# Autodesk Inventor assembly: Passion-v2
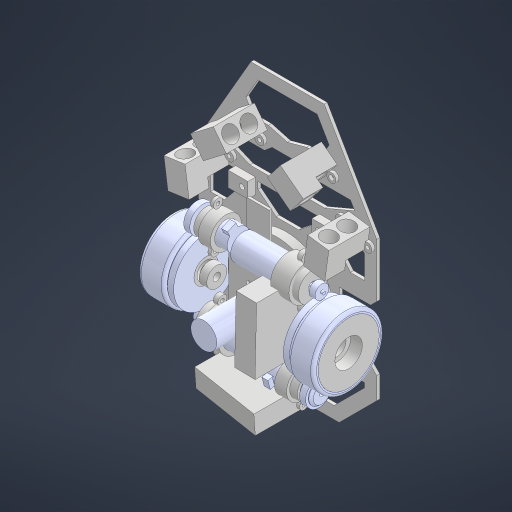
[picture p0: Inventor's stored thumbnail of the model, 512x512]
Saved by Autodesk Inventor 2023.5 (Build 275446000, 446)
## iProperties
Created: 2025-01-19
Part Number: Passion-v2
Document SubType Name: Assembly
Designer: IshiiLabHonda
Author: IshiiLabHonda
## Documents named in this file (20)
- C:\Users\IshiiLabHonda\Documents\Micromouse\Passion-v2\Inventor\Passion-v2-2\Passion-v2.iam
- C:\Users\IshiiLabHonda\Documents\Micromouse\Passion-v2\Inventor\Passion-v2-2\Origin\fan.ipt
- C:\Users\IshiiLabHonda\Documents\Micromouse\Passion-v2\Inventor\Passion-v2-2\Origin\chassis.ipt
- C:\Users\IshiiLabHonda\Documents\Micromouse\Passion-v2\Inventor\Passion-v2-2\Readymade\Motor-8520.ipt
- C:\Users\IshiiLabHonda\Documents\Micromouse\Passion-v2\Inventor\Passion-v2-2\Readymade\Encoder-7S-400-2MC-50-00E.ipt
- C:\Users\IshiiLabHonda\Documents\Micromouse\Passion-v2\Inventor\Passion-v2-2\Readymade\Pinion-Gear_M0.3_15T.ipt
- C:\Users\IshiiLabHonda\Documents\Micromouse\Passion-v2\Inventor\Passion-v2-2\Readymade\Encoder-Gear_M0.3_29T.ipt
- C:\Users\IshiiLabHonda\Documents\Micromouse\Passion-v2\Inventor\Passion-v2-2\Readymade\Spur-Gear_M0.3_71T_t2.0_D8.ipt
- C:\Users\IshiiLabHonda\Documents\Micromouse\Passion-v2\Inventor\Passion-v2-2\Readymade\Wheel_MZH131W-N2.ipt
- C:\Users\IshiiLabHonda\Documents\Micromouse\Passion-v2\Inventor\Passion-v2-2\Readymade\Tire-MZW39-40.ipt
- C:\Users\IshiiLabHonda\Documents\Micromouse\Passion-v2\Inventor\Passion-v2-2\Readymade\Encoder-Gear-Spacer.ipt
- C:\Users\IshiiLabHonda\Documents\Micromouse\Passion-v2\Inventor\Passion-v2-2\Origin\motormount-r.ipt
- C:\Users\IshiiLabHonda\Documents\Micromouse\Passion-v2\Inventor\Passion-v2-2\Origin\motormount-l.ipt
- C:\Users\IshiiLabHonda\Documents\Micromouse\Passion-v2\Inventor\Passion-v2-2\Common\spacer-outwheel-m3-1.ipt
- C:\Users\IshiiLabHonda\Documents\Micromouse\Passion-v2\Inventor\Passion-v2-2\Origin\circuit.ipt
- C:\Users\IshiiLabHonda\Documents\Micromouse\Passion-v2\Inventor\Passion-v2-2\Origin\encodersupporter.ipt
- C:\Users\IshiiLabHonda\Documents\Micromouse\Passion-v2\Inventor\Passion-v2-2\Origin\sensormount.ipt
- C:\Users\IshiiLabHonda\Documents\Micromouse\Passion-v2\Inventor\Passion-v2-2\Origin\sensormount-2.ipt
- C:\Users\IshiiLabHonda\Documents\Micromouse\Passion-v2\Inventor\Passion-v2-2\Readymade\Lipo-1C-FX100C.ipt
- C:\Users\IshiiLabHonda\Documents\Micromouse\Passion-v2\Inventor\Passion-v2-2\Origin\motorsupporter.ipt
## Components (32 placed, 19 different names)
1. fan:1 — メイト:7, メイト:52, 角度:5
2. chassis:1 — フラッシュ:1, メイト:1, メイト:2, メイト:7, メイト:37, メイト:43, メイト:71, メイト:74, 角度:3, メイト:78, メイト:79, メイト:80, メイト:81, メイト:82, 角度:4, メイト:86
3. Motor-8520:1 — メイト:12, メイト:44, メイト:45, メイト:87
4. Encoder-7S-400-2MC-50-00E:1 — メイト:13, メイト:50, メイト:51, メイト:61
5. Pinion-Gear_M0.3_15T:1 — メイト:12, フラッシュ:7
6. Encoder-Gear_M0.3_29T:1 — メイト:13, メイト:18, メイト:19, フラッシュ:6
7. Spur-Gear_M0.3_71T_t2.0_D8:1 — メイト:17, メイト:59, フラッシュ:6, フラッシュ:7
8. Wheel_MZH131W-N2:1 — メイト:15, フラッシュ:2, メイト:17, メイト:56, メイト:59, メイト:60
9. Tire-MZW39-40:1 — メイト:15, フラッシュ:2
10. Encoder-Gear-Spacer:1 — メイト:18, メイト:19
11. motormount-r:1 — メイト:37, メイト:38, メイト:39, メイト:40, メイト:47, メイト:49, メイト:67, メイト:80, メイト:81
12. Encoder-7S-400-2MC-50-00E:2 — メイト:34, メイト:39, メイト:49, メイト:65
13. Motor-8520:2 — メイト:33, メイト:40, メイト:88
14. Spur-Gear_M0.3_71T_t2.0_D8:2 — メイト:29, フラッシュ:4, フラッシュ:5
15. Wheel_MZH131W-N2:2 — メイト:29, メイト:38, メイト:48
16. Tire-MZW39-40:2 — メイト:46
17. Pinion-Gear_M0.3_15T:2 — メイト:33, フラッシュ:4
18. Encoder-Gear_M0.3_29T:2 — メイト:34, フラッシュ:5
19. Encoder-Gear-Spacer:2
20. motormount-l:1 — メイト:43, メイト:44, メイト:45, メイト:50, メイト:51, メイト:57, メイト:58, メイト:62, メイト:78, メイト:79
21. spacer-outwheel-m3-1:1 — メイト:46, メイト:47, メイト:48
22. Motor-8520:3 — メイト:52, 正接:2, メイト:82, メイト:83
23. circuit:1 — メイト:83, 角度:4, メイト:86
24. spacer-outwheel-m3-1:2 — メイト:56, メイト:57, メイト:58, メイト:60
25. encodersupporter:1 — メイト:61, メイト:62
26. encodersupporter:4 — メイト:65, メイト:67
27. sensormount:1 — メイト:71
28. sensormount-2:1 — メイト:74
29. Lipo-1C-FX100C:1 — 角度:3, 正接:2
30. Lipo-1C-FX100C:3
31. motorsupporter:1 — メイト:87
32. motorsupporter:2 — メイト:88, 角度:5
## Relationships (61: Mate 50, Flush 7, Angle 3, Tangent 1)
- フラッシュ:1 [Flush]: chassis:1
- メイト:1 [Mate]: chassis:1
- メイト:2 [Mate]: chassis:1
- メイト:7 [Mate] (0.5 mm): fan:1 ↔ chassis:1
- メイト:12 [Mate]: Motor-8520:1 ↔ Pinion-Gear_M0.3_15T:1
- メイト:13 [Mate]: Encoder-7S-400-2MC-50-00E:1 ↔ Encoder-Gear_M0.3_29T:1
- メイト:15 [Mate]: Wheel_MZH131W-N2:1 ↔ Tire-MZW39-40:1
- フラッシュ:2 [Flush]: Wheel_MZH131W-N2:1 ↔ Tire-MZW39-40:1
- メイト:17 [Mate]: Spur-Gear_M0.3_71T_t2.0_D8:1 ↔ Wheel_MZH131W-N2:1
- メイト:18 [Mate]: Encoder-Gear_M0.3_29T:1 ↔ Encoder-Gear-Spacer:1
- メイト:19 [Mate]: Encoder-Gear_M0.3_29T:1 ↔ Encoder-Gear-Spacer:1
- [Mate]: Wheel_MZH131W-N2:2 ↔ Tire-MZW39-40:2
- [Flush]: Wheel_MZH131W-N2:2 ↔ Tire-MZW39-40:2
- [Mate]: Spur-Gear_M0.3_71T_t2.0_D8:2 ↔ Wheel_MZH131W-N2:2
- メイト:29 [Mate]: Spur-Gear_M0.3_71T_t2.0_D8:2 ↔ Wheel_MZH131W-N2:2
- [Mate]: Encoder-Gear_M0.3_29T:2 ↔ Encoder-Gear-Spacer:2
- [Mate]: Encoder-Gear_M0.3_29T:2 ↔ Encoder-Gear-Spacer:2
- メイト:33 [Mate]: Motor-8520:2 ↔ Pinion-Gear_M0.3_15T:2
- メイト:34 [Mate]: Encoder-7S-400-2MC-50-00E:2 ↔ Encoder-Gear_M0.3_29T:2
- メイト:37 [Mate]: chassis:1 ↔ motormount-r:1
- メイト:38 [Mate]: motormount-r:1 ↔ Wheel_MZH131W-N2:2
- メイト:39 [Mate]: motormount-r:1 ↔ Encoder-7S-400-2MC-50-00E:2
- メイト:40 [Mate]: motormount-r:1 ↔ Motor-8520:2
- メイト:43 [Mate]: chassis:1 ↔ motormount-l:1
- メイト:44 [Mate]: Motor-8520:1 ↔ motormount-l:1
- メイト:45 [Mate]: Motor-8520:1 ↔ motormount-l:1
- メイト:46 [Mate]: Tire-MZW39-40:2 ↔ spacer-outwheel-m3-1:1
- メイト:47 [Mate]: motormount-r:1 ↔ spacer-outwheel-m3-1:1
- メイト:48 [Mate]: Wheel_MZH131W-N2:2 ↔ spacer-outwheel-m3-1:1
- フラッシュ:4 [Flush]: Spur-Gear_M0.3_71T_t2.0_D8:2 ↔ Pinion-Gear_M0.3_15T:2
- フラッシュ:5 [Flush]: Spur-Gear_M0.3_71T_t2.0_D8:2 ↔ Encoder-Gear_M0.3_29T:2
- メイト:49 [Mate]: motormount-r:1 ↔ Encoder-7S-400-2MC-50-00E:2
- メイト:50 [Mate]: Encoder-7S-400-2MC-50-00E:1 ↔ motormount-l:1
- メイト:51 [Mate]: Encoder-7S-400-2MC-50-00E:1 ↔ motormount-l:1
- メイト:52 [Mate]: fan:1 ↔ Motor-8520:3
- メイト:56 [Mate]: Wheel_MZH131W-N2:1 ↔ spacer-outwheel-m3-1:2
- メイト:57 [Mate]: motormount-l:1 ↔ spacer-outwheel-m3-1:2
- メイト:58 [Mate]: motormount-l:1 ↔ spacer-outwheel-m3-1:2
- メイト:59 [Mate]: Spur-Gear_M0.3_71T_t2.0_D8:1 ↔ Wheel_MZH131W-N2:1
- メイト:60 [Mate]: Wheel_MZH131W-N2:1 ↔ spacer-outwheel-m3-1:2
- メイト:61 [Mate]: Encoder-7S-400-2MC-50-00E:1 ↔ encodersupporter:1
- メイト:62 [Mate]: motormount-l:1 ↔ encodersupporter:1
- メイト:65 [Mate]: Encoder-7S-400-2MC-50-00E:2 ↔ encodersupporter:4
- メイト:67 [Mate]: motormount-r:1 ↔ encodersupporter:4
- メイト:71 [Mate]: chassis:1 ↔ sensormount:1
- メイト:74 [Mate]: chassis:1 ↔ sensormount-2:1
- 角度:3 [Angle] (0 deg): chassis:1 ↔ Lipo-1C-FX100C:1
- 正接:2 [Tangent]: Motor-8520:3 ↔ Lipo-1C-FX100C:1
- メイト:78 [Mate]: chassis:1 ↔ motormount-l:1
- メイト:79 [Mate]: chassis:1 ↔ motormount-l:1
- メイト:80 [Mate]: chassis:1 ↔ motormount-r:1
- メイト:81 [Mate]: chassis:1 ↔ motormount-r:1
- メイト:82 [Mate]: chassis:1 ↔ Motor-8520:3
- フラッシュ:6 [Flush]: Encoder-Gear_M0.3_29T:1 ↔ Spur-Gear_M0.3_71T_t2.0_D8:1
- フラッシュ:7 [Flush]: Pinion-Gear_M0.3_15T:1 ↔ Spur-Gear_M0.3_71T_t2.0_D8:1
- メイト:83 [Mate]: Motor-8520:3 ↔ circuit:1
- 角度:4 [Angle] (0 deg): chassis:1 ↔ circuit:1
- メイト:86 [Mate] (4.5 mm): chassis:1 ↔ circuit:1
- メイト:87 [Mate]: Motor-8520:1 ↔ motorsupporter:1
- メイト:88 [Mate]: Motor-8520:2 ↔ motorsupporter:2
- 角度:5 [Angle] (180 deg): fan:1 ↔ motorsupporter:2
## Named parameters: d41_d25 = 0 mm, d42_d26 = 0 mm, d43_d28 = 0 mm, d46_d29 = 0 mm, d47_d30 = 0 mm
